# Autodesk Inventor assembly: ASY ДМФ 0100 Барабан v2.1
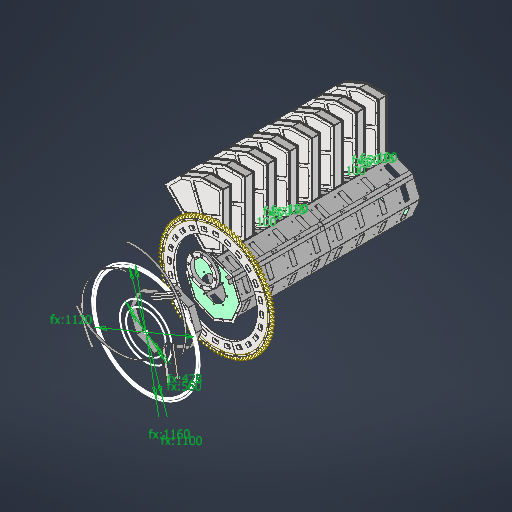
[picture p0: Inventor's stored thumbnail of the model, 512x512]
Saved by Autodesk Inventor 2026.2 (Build 302298000, 298)
## iProperties
Created: 2024-04-28
Part Number: ASY ДМФ 0100 Барабан v2.1
Document SubType Name: Assembly
Designer: pokla
Author: pokla
## Documents named in this file (29)
- C:\Users\admin\Documents\Inventor\DMF-Disk-Micro-Filter\Барабан v2.1\ASY ДМФ 0100 Барабан v2.1.iam
- C:\Users\admin\Documents\Inventor\DMF-Disk-Micro-Filter\Барабан v2.1\DMF 01 21 Барабан торец НОС v2.1.ipt
- C:\Users\admin\Documents\Inventor\DMF-Disk-Micro-Filter\Барабан v2.1\DMF 01 13 Барабан Лист лев брт v2.1.ipt
- C:\Users\admin\Documents\Inventor\DMF-Disk-Micro-Filter\Барабан v2.1\DMF 01 14 Барабан Лист прав брт v2.1.ipt
- C:\Users\admin\Documents\Inventor\DMF-Disk-Micro-Filter\Барабан v2.1\DMF 01 31 Барабан Опорное кольцо НОС v2.1.ipt
- C:\Users\admin\Documents\Inventor\DMF-Disk-Micro-Filter\Барабан v2.1\DMF 01 17 опора крышки v2.1.ipt
- C:\Users\admin\Documents\Inventor\DMF-Disk-Micro-Filter\Барабан v2.1\DMF 000 размеры v2.1.ipt
- C:\Users\admin\Documents\Inventor\DMF-Disk-Micro-Filter\Барабан v2.1\DMF 01 12 Барабан усилитель v2.1.ipt
- C:\Users\admin\Documents\Inventor\DMF-Disk-Micro-Filter\Барабан v2.1\ASY DMF 010 cap v2.1.iam
- C:\Users\admin\Documents\Inventor\DMF-Disk-Micro-Filter\Барабан v2.1\DMF 01 32 Барабан Опорное кольцо КОРМА v2.1.ipt
- C:\Users\admin\Documents\Inventor\DMF-Disk-Micro-Filter\Барабан v2.1\DMF 01 22 Барабан торец КОРМА v2.1.ipt
- C:\Users\admin\Documents\Inventor\DMF-Disk-Micro-Filter\Барабан v2.1\ASY DMF filter package v2.1.iam
- C:\Users\admin\Documents\Inventor\DMF-Disk-Micro-Filter\Барабан v2.1\DMF 01 21 cylinder butt end nose.ipt
- C:\Users\admin\Documents\Inventor\DMF-Disk-Micro-Filter\Барабан v2.1\DMF 2.1 01 42 Gear way 2.ipt
- C:\Users\admin\Documents\Inventor\DMF-Disk-Micro-Filter\Барабан v2.1\DMF 2.1 01 43 Gear rim 3.ipt
- C:\Users\admin\Documents\Inventor\DMF-Disk-Micro-Filter\Барабан v2.1\DMF 2.1 01 44 Gear rim 4.ipt
- C:\Users\admin\Documents\Inventor\DMF-Disk-Micro-Filter\Барабан v2.1\DMF 2.1 01 45 Gear ring 5.ipt
- C:\Users\admin\Documents\Inventor\DMF-Disk-Micro-Filter\Барабан v2.1\DMF 2.1 01 46 Gear axis wheel 6.ipt
- C:\Users\admin\Documents\Inventor\DMF-Disk-Micro-Filter\Барабан v2.1\DMF 01 13 Барабан усилитель v2.1.ipt
- C:\Users\admin\Documents\Inventor\DMF-Disk-Micro-Filter\шестерни 06.09.2025\DMF sector big gear 2.1.ipt
- C:\Users\admin\Documents\Inventor\DMF-Disk-Micro-Filter\Барабан v2.1\DMF 01 15 drum sheet 1.ipt
- C:\Users\admin\Documents\Inventor\DMF-Disk-Micro-Filter\ДМФ 01 12 Барабан усилитель.ipt
- C:\Users\admin\Documents\Inventor\DMF-Disk-Micro-Filter\ДМФ 01 15 Барабан усилитель борта.ipt
- C:\Users\admin\Documents\Inventor\DMF-Disk-Micro-Filter\Барабан v2.1\DMF 2.1 Пластина паза маленькая.ipt
- C:\Users\admin\Documents\Inventor\DMF-Disk-Micro-Filter\Барабан v2.1\DMF 2.1 Пластина паза большая.ipt
- C:\Users\admin\Documents\Inventor\DMF-Disk-Micro-Filter\Барабан v2.1\DMF 01 14 Барабан Лист прав брт №2 v2.1.ipt
- C:\Users\admin\Documents\Inventor\DMF-Disk-Micro-Filter\Барабан v2.1\DMF 01 13 Барабан Лист лев брт №2 v2.1.ipt
- C:\Users\admin\Documents\Inventor\DMF-Disk-Micro-Filter\Барабан v2.1\ASY DMF 010 cap №2 v2.1.iam
- C:\Users\admin\Documents\Inventor\DMF-Disk-Micro-Filter\Барабан v2.1\DMF 01 17 опора крышки v2.1_CPY.ipt
## Components (97 placed, 34 different names)
1. DMF 000 размеры v2.1.ipt:1
2. DMF 01 21 Барабан торец НОС v2.1.ipt:1 — Rigid:81, Rigid:94
3. DMF 01 31 Барабан Опорное кольцо НОС v2.1.ipt:1
4. DMF 01 32 Барабан Опорное кольцо КОРМА v2.1.ipt:1 — Rigid:20
5. DMF 01 22 Барабан торец КОРМА v2.1.ipt:1 — Rigid:20, Rigid:51, Rigid:53, Mate:36, Flush:22, Flush:23, Mate:37, Flush:24, Flush:25, Mate:45, Flush:34, Flush:35
6. DMF 01 13 Барабан Лист лев брт v2.1.ipt:1 — Rigid:51, Rigid:86
7. DMF 01 14 Барабан Лист прав брт v2.1.ipt:1 — Rigid:53, Rigid:85
8. DMF 01 17 опора крышки v2.1.ipt:1 — Mate:37, Flush:24, Flush:25, Rigid:93
9. DMF 01 17 опора крышки v2.1.ipt:2 — Mate:36, Flush:22, Flush:23, Rigid:92
10. ASY DMF 010 cap v2.1.iam:1 [sub-assembly] — Mate:45, Flush:34, Flush:35, Rigid:84, Rigid:90, Rigid:91
11. DMF 01 21 cylinder butt end nose.ipt:1
12. DMF 2.1 01 45 Gear ring 5.ipt:1
13. DMF 2.1 01 46 Gear axis wheel 6.ipt:1
14. DMF 2.1 01 44 Gear rim 4.ipt:1
15. DMF 2.1 01 43 Gear rim 3.ipt:2 — Rigid:24, Rigid:35
16. DMF 2.1 01 43 Gear rim 3.ipt:1 — Rigid:24
17. DMF 2.1 01 43 Gear rim 3.ipt:3 — Rigid:35, Rigid:36
18. DMF 2.1 01 43 Gear rim 3.ipt:4
19. DMF 2.1 01 43 Gear rim 3.ipt:5 — Rigid:36, Rigid:38, Rigid:81
20. DMF 2.1 01 43 Gear rim 3.ipt:6 — Rigid:42
21. DMF 2.1 01 43 Gear rim 3.ipt:7 — Rigid:38
22. DMF 2.1 01 43 Gear rim 3.ipt:8
23. DMF 2.1 01 44 Gear rim 4.ipt:2
24. DMF 2.1 01 44 Gear rim 4.ipt:3
25. DMF 01 15 drum sheet 1.ipt:1
26. DMF 01 15 drum sheet 1.ipt:2
27. ДМФ 01 12 Барабан усилитель.ipt:2 — Rigid:56, Rigid:57, Rigid:89
28. ДМФ 01 15 Барабан усилитель борта.ipt:3 — Rigid:56
29. ДМФ 01 15 Барабан усилитель борта.ipt:4 — Rigid:57
30. DMF 01 14 Барабан Лист прав брт №2 v2.1:1 — Rigid:85, Rigid:94
31. DMF 01 13 Барабан Лист лев брт №2 v2.1:1 — Rigid:86
32. ASY DMF 010 cap №2 v2.1:1 [sub-assembly] — Rigid:84, Flush:40, Mate:52, Mate:53
33. ДМФ 01 12 Барабан усилитель:3 — Flush:40, Mate:52, Mate:53, Rigid:89
34. ДМФ 01 15 Барабан усилитель борта:5
35. ДМФ 01 15 Барабан усилитель борта:6
36. DMF 01 17 опора крышки №2 v2.1:1 — Rigid:92
37. DMF 01 17 опора крышки №2 v2.1:2 — Rigid:93
38. DMF 01 12 Барабан усилитель v2.1.ipt:1 — Rigid:82
39. DMF 01 13 Барабан усилитель v2.1.ipt:1 — Rigid:82
40. DMF 01 12 Барабан усилитель v2.1.ipt:2
41. DMF 01 13 Барабан усилитель v2.1.ipt:2
42. ASY DMF filter package v2.1.iam:1 [sub-assembly] — Rigid:59
43. DMF 2.1 01 42 Gear way 2.ipt:1 — Rigid:59, Rigid:91
44. DMF 2.1 Пластина паза большая:1 — Rigid:62
45. DMF 2.1 Пластина паза маленькая.ipt:1 — Rigid:62, Rigid:90
46. ASY DMF filter package v2.1:2 [sub-assembly]
47. DMF 2.1 01 42 Gear way 2:2
48. DMF 2.1 Пластина паза большая:2
49. DMF 2.1 Пластина паза маленькая:2
50. ASY DMF filter package v2.1:3 [sub-assembly]
51. DMF 2.1 01 42 Gear way 2:3
52. DMF 2.1 Пластина паза большая:3
53. DMF 2.1 Пластина паза маленькая:3
54. ASY DMF filter package v2.1:4 [sub-assembly]
55. DMF 2.1 01 42 Gear way 2:4
56. DMF 2.1 Пластина паза большая:4
57. DMF 2.1 Пластина паза маленькая:4
58. ASY DMF filter package v2.1:5 [sub-assembly]
59. DMF 2.1 01 42 Gear way 2:5
60. DMF 2.1 Пластина паза большая:5
61. DMF 2.1 Пластина паза маленькая:5
62. ASY DMF filter package v2.1:6 [sub-assembly]
63. DMF 2.1 01 42 Gear way 2:6
64. DMF 2.1 Пластина паза большая:6
65. DMF 2.1 Пластина паза маленькая:6
66. ASY DMF filter package v2.1:7 [sub-assembly]
67. DMF 2.1 01 42 Gear way 2:7
68. DMF 2.1 Пластина паза большая:7
69. DMF 2.1 Пластина паза маленькая:7
70. ASY DMF filter package v2.1:8 [sub-assembly]
71. DMF 2.1 01 42 Gear way 2:8
72. DMF 2.1 Пластина паза большая:8
73. DMF 2.1 Пластина паза маленькая:8
74. DMF sector big gear 2.1.ipt:1 — Rigid:42
75. DMF sector big gear 2.1:2
76. DMF sector big gear 2.1:3
77. DMF sector big gear 2.1:4
78. DMF sector big gear 2.1:5
79. DMF sector big gear 2.1:6
80. DMF sector big gear 2.1:7
81. DMF sector big gear 2.1:8
82. DMF sector big gear 2.1:9
83. DMF sector big gear 2.1:10
84. DMF sector big gear 2.1:11
85. DMF sector big gear 2.1:12
86. DMF sector big gear 2.1:13
87. DMF sector big gear 2.1:14
88. DMF sector big gear 2.1:15
89. DMF sector big gear 2.1:16
90. DMF sector big gear 2.1:17
91. DMF sector big gear 2.1:18
92. DMF sector big gear 2.1:19
93. DMF sector big gear 2.1:20
94. DMF sector big gear 2.1:21
95. DMF sector big gear 2.1:22
96. DMF sector big gear 2.1:23
97. DMF sector big gear 2.1:24
## Component patterns: (8 elements, first: ASY DMF filter package v2.1.iam:1 + DMF 2.1 01 42 Gear way 2.ipt:1 + DMF 2.1 Пластина паза большая:1 + DMF 2.1 Пластина паза маленькая.ipt:1), (24 elements, first: DMF sector big gear 2.1.ipt:1)
## Relationships (40: WeldJoint 28, Flush 7, Mate 5)
- Rigid:20 [WeldJoint]: DMF 01 32 Барабан Опорное кольцо КОРМА v2.1.ipt:1 ↔ DMF 01 22 Барабан торец КОРМА v2.1.ipt:1
- Rigid:24 [WeldJoint] (25 mm): DMF 2.1 01 43 Gear rim 3.ipt:2 ↔ DMF 2.1 01 43 Gear rim 3.ipt:1
- [WeldJoint] (25 mm): DMF 2.1 01 43 Gear rim 3.ipt:3 ↔ DMF 2.1 01 43 Gear rim 3.ipt:4
- [WeldJoint] (25 mm): DMF 2.1 01 43 Gear rim 3.ipt:5 ↔ DMF 2.1 01 43 Gear rim 3.ipt:6
- Rigid:35 [WeldJoint]: DMF 2.1 01 43 Gear rim 3.ipt:2 ↔ DMF 2.1 01 43 Gear rim 3.ipt:3
- Rigid:36 [WeldJoint]: DMF 2.1 01 43 Gear rim 3.ipt:3 ↔ DMF 2.1 01 43 Gear rim 3.ipt:5
- [WeldJoint] (25 mm): DMF 2.1 01 43 Gear rim 3.ipt:7 ↔ DMF 2.1 01 43 Gear rim 3.ipt:8
- Rigid:38 [WeldJoint]: DMF 2.1 01 43 Gear rim 3.ipt:5 ↔ DMF 2.1 01 43 Gear rim 3.ipt:7
- Rigid:42 [WeldJoint]: DMF 2.1 01 43 Gear rim 3.ipt:6 ↔ DMF sector big gear 2.1.ipt:1
- Rigid:51 [WeldJoint]: DMF 01 22 Барабан торец КОРМА v2.1.ipt:1 ↔ DMF 01 13 Барабан Лист лев брт v2.1.ipt:1
- Rigid:53 [WeldJoint]: DMF 01 22 Барабан торец КОРМА v2.1.ipt:1 ↔ DMF 01 14 Барабан Лист прав брт v2.1.ipt:1
- Mate:36: DMF 01 22 Барабан торец КОРМА v2.1.ipt:1 ↔ DMF 01 17 опора крышки v2.1.ipt:2
- Flush:22 (2 mm): DMF 01 22 Барабан торец КОРМА v2.1.ipt:1 ↔ DMF 01 17 опора крышки v2.1.ipt:2
- Flush:23 (2 mm): DMF 01 22 Барабан торец КОРМА v2.1.ipt:1 ↔ DMF 01 17 опора крышки v2.1.ipt:2
- Mate:37: DMF 01 22 Барабан торец КОРМА v2.1.ipt:1 ↔ DMF 01 17 опора крышки v2.1.ipt:1
- Flush:24 (2 mm): DMF 01 22 Барабан торец КОРМА v2.1.ipt:1 ↔ DMF 01 17 опора крышки v2.1.ipt:1
- Flush:25 (2 mm): DMF 01 22 Барабан торец КОРМА v2.1.ipt:1 ↔ DMF 01 17 опора крышки v2.1.ipt:1
- Rigid:56 [WeldJoint]: ДМФ 01 12 Барабан усилитель.ipt:2 ↔ ДМФ 01 15 Барабан усилитель борта.ipt:3
- Rigid:57 [WeldJoint]: ДМФ 01 12 Барабан усилитель.ipt:2 ↔ ДМФ 01 15 Барабан усилитель борта.ipt:4
- Mate:45: DMF 01 22 Барабан торец КОРМА v2.1.ipt:1 ↔ ASY DMF 010 cap v2.1.iam:1
- Flush:34: DMF 01 22 Барабан торец КОРМА v2.1.ipt:1 ↔ ASY DMF 010 cap v2.1.iam:1
- Flush:35: DMF 01 22 Барабан торец КОРМА v2.1.ipt:1 ↔ ASY DMF 010 cap v2.1.iam:1
- Rigid:59 [WeldJoint] (5 mm): ASY DMF filter package v2.1.iam:1 ↔ DMF 2.1 01 42 Gear way 2.ipt:1
- Rigid:62 [WeldJoint]: DMF 2.1 Пластина паза большая:1 ↔ DMF 2.1 Пластина паза маленькая.ipt:1
- Rigid:81 [WeldJoint] (-20.5 mm): DMF 01 21 Барабан торец НОС v2.1.ipt:1 ↔ DMF 2.1 01 43 Gear rim 3.ipt:5
- Rigid:82 [WeldJoint]: DMF 01 12 Барабан усилитель v2.1.ipt:1 ↔ DMF 01 13 Барабан усилитель v2.1.ipt:1
- Rigid:84 [WeldJoint]: ASY DMF 010 cap v2.1.iam:1 ↔ ASY DMF 010 cap №2 v2.1:1
- Rigid:85 [WeldJoint]: DMF 01 14 Барабан Лист прав брт v2.1.ipt:1 ↔ DMF 01 14 Барабан Лист прав брт №2 v2.1:1
- Rigid:86 [WeldJoint]: DMF 01 13 Барабан Лист лев брт v2.1.ipt:1 ↔ DMF 01 13 Барабан Лист лев брт №2 v2.1:1
- [WeldJoint]: ДМФ 01 12 Барабан усилитель:3 ↔ ДМФ 01 15 Барабан усилитель борта:5
- [WeldJoint]: ДМФ 01 12 Барабан усилитель:3 ↔ ДМФ 01 15 Барабан усилитель борта:6
- Flush:40: ASY DMF 010 cap №2 v2.1:1 ↔ ДМФ 01 12 Барабан усилитель:3
- Mate:52: ASY DMF 010 cap №2 v2.1:1 ↔ ДМФ 01 12 Барабан усилитель:3
- Mate:53: ASY DMF 010 cap №2 v2.1:1 ↔ ДМФ 01 12 Барабан усилитель:3
- Rigid:89 [WeldJoint]: ДМФ 01 12 Барабан усилитель.ipt:2 ↔ ДМФ 01 12 Барабан усилитель:3
- Rigid:90 [WeldJoint] (-48.5 mm): ASY DMF 010 cap v2.1.iam:1 ↔ DMF 2.1 Пластина паза маленькая.ipt:1
- Rigid:91 [WeldJoint]: ASY DMF 010 cap v2.1.iam:1 ↔ DMF 2.1 01 42 Gear way 2.ipt:1
- Rigid:92 [WeldJoint]: DMF 01 17 опора крышки v2.1.ipt:2 ↔ DMF 01 17 опора крышки №2 v2.1:1
- Rigid:93 [WeldJoint]: DMF 01 17 опора крышки v2.1.ipt:1 ↔ DMF 01 17 опора крышки №2 v2.1:2
- Rigid:94 [WeldJoint]: DMF 01 21 Барабан торец НОС v2.1.ipt:1 ↔ DMF 01 14 Барабан Лист прав брт №2 v2.1:1
## Named parameters: d314_d251 = 25 mm, d315_d251 = 25 mm, d318_d251 = 25 mm, d460_d378 = 0 mm, d461_d379 = 0 mm
